# Autodesk Inventor assembly: Y_Carriage_V2
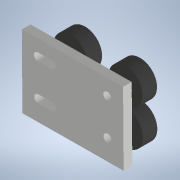
[picture p0: Inventor's stored thumbnail of the model, 180x180]
Saved by Autodesk Inventor 2021 (Build 250183000, 183)
## iProperties
Created: 2021-06-15
Part Number: Y_Carriage_V2
Document SubType Name: Assembly
Designer: Jorian Brusind
Author: Jorian Brusind
## Documents named in this file (4)
- C:\Users\Jorian Brusind\Documents\GitHub\PersonalProjects\HyperRail\Inventor Files\Y_Carriage_V2.iam
- C:\Users\Jorian Brusind\Documents\GitHub\PersonalProjects\HyperRail\Inventor Files\11mm_BearingWheel.ipt
- C:\Users\Jorian Brusind\Documents\GitHub\PersonalProjects\HyperRail\Inventor Files\6mm_Spacer.ipt
- C:\Users\Jorian Brusind\Documents\GitHub\PersonalProjects\HyperRail\Inventor Files\Y_Carriage_Plate.ipt
## Components (9 placed, 3 different names)
1. 11mm_BearingWheel:1 — Mate:5, Mate:6, Mate:8, Flush:1
2. 11mm_BearingWheel:2 — Mate:10, Flush:2, Mate:14
3. 11mm_BearingWheel:3 — Mate:1, Mate:2, Mate:4
4. 11mm_BearingWheel:4 — Mate:9, Flush:1, Flush:2, Mate:12
5. 6mm_Spacer:1 — Mate:13, Mate:14
6. 6mm_Spacer:2 — Mate:6, Mate:7, Mate:8
7. 6mm_Spacer:3 — Mate:3, Mate:4
8. 6mm_Spacer:4 — Mate:11, Mate:12
9. Y_Carriage_Plate:1 — Mate:1, Mate:2, Mate:3, Mate:5, Mate:7, Mate:9, Mate:10, Mate:11, Mate:13
## Relationships (16: Mate 14, Flush 2)
- Mate:1: 11mm_BearingWheel:3 ↔ Y_Carriage_Plate:1
- Mate:2 (6 mm): 11mm_BearingWheel:3 ↔ Y_Carriage_Plate:1
- Mate:3: 6mm_Spacer:3 ↔ Y_Carriage_Plate:1
- Mate:4: 11mm_BearingWheel:3 ↔ 6mm_Spacer:3
- Mate:5: 11mm_BearingWheel:1 ↔ Y_Carriage_Plate:1
- Mate:6: 11mm_BearingWheel:1 ↔ 6mm_Spacer:2
- Mate:7: 6mm_Spacer:2 ↔ Y_Carriage_Plate:1
- Mate:8: 11mm_BearingWheel:1 ↔ 6mm_Spacer:2
- Mate:9: 11mm_BearingWheel:4 ↔ Y_Carriage_Plate:1
- Mate:10: 11mm_BearingWheel:2 ↔ Y_Carriage_Plate:1
- Flush:1: 11mm_BearingWheel:1 ↔ 11mm_BearingWheel:4
- Flush:2: 11mm_BearingWheel:2 ↔ 11mm_BearingWheel:4
- Mate:11: 6mm_Spacer:4 ↔ Y_Carriage_Plate:1
- Mate:12: 11mm_BearingWheel:4 ↔ 6mm_Spacer:4
- Mate:13: 6mm_Spacer:1 ↔ Y_Carriage_Plate:1
- Mate:14: 11mm_BearingWheel:2 ↔ 6mm_Spacer:1
